# Autodesk Inventor assembly: 1.625_flex_wheel_w_versahex
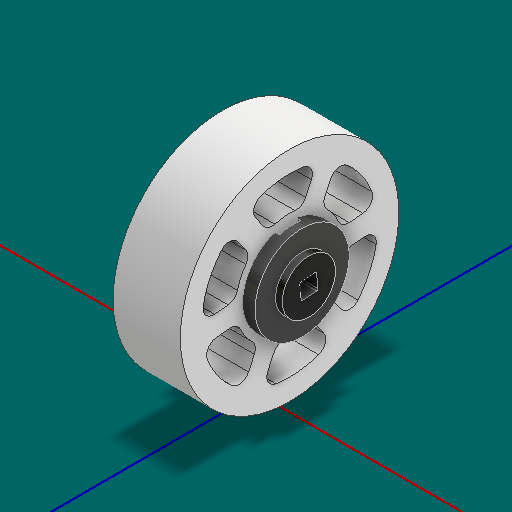
[picture p0: Inventor's stored thumbnail of the model, 512x512]
Saved by Autodesk Inventor 2025 (Build 290162000, 162)
## iProperties
Created: 2024-08-18
Part Number: 1.625_flex_wheel_w_versahex
Document SubType Name: Assembly
Designer: averey
Author: averey
## Documents named in this file (5)
- C:\Users\avere\vex_robotics_high_stakes\hardware\cad\_quick_assemblies\1.625_flex_wheel_w_versahex.iam
- C:\Users\avere\vex_robotics_high_stakes\hardware\cad\VEX-CAD-Inventor\Motion\Wheels\Flex Wheels\1.625 Flex Wheel\1.625 30A .500.ipt
- C:\Users\avere\vex_robotics_high_stakes\hardware\cad\VEX-CAD-Inventor\Motion\Wheels\Flex Wheels\1.625 Flex Wheel.ipt
- C:\Users\avere\vex_robotics_high_stakes\hardware\cad\VEX-CAD-Inventor\Motion\Wheels\Flex Wheels\VersaHex Adapters .125.ipt
- C:\Users\avere\vex_robotics_high_stakes\hardware\cad\VEX-CAD-Inventor\Motion\Insert Square.ipt
## Components (5 placed, 3 different names)
1. 1.625 30A .500:1 — Mate:1, Mate:2, Mate:3, Angle:5
2. VersaHex Adapters .125:1
3. Insert Square:1
4. VersaHex Adapters .125:2
5. Insert Square:2
## Relationships (12: Angle 5, Insert 4, Mate 3)
- [Insert]: VersaHex Adapters .125:1 ↔ Insert Square:1
- [Angle] (0 deg): VersaHex Adapters .125:1 ↔ Insert Square:1
- [Angle] (0 deg): 1.625 30A .500:1 ↔ VersaHex Adapters .125:1
- [Insert]: 1.625 30A .500:1 ↔ VersaHex Adapters .125:1
- [Insert]: VersaHex Adapters .125:2 ↔ Insert Square:2
- [Angle] (0 deg): VersaHex Adapters .125:2 ↔ Insert Square:2
- [Angle] (0 deg): 1.625 30A .500:1 ↔ VersaHex Adapters .125:2
- [Insert]: 1.625 30A .500:1 ↔ VersaHex Adapters .125:2
- Mate:1: 1.625 30A .500:1
- Mate:2 (6.35 mm): 1.625 30A .500:1
- Mate:3: 1.625 30A .500:1
- Angle:5 (0 deg): 1.625 30A .500:1
## Named parameters: d0_d5 = 0 mm, d1_d6 = 0 deg, d2_d7 = 0 deg, d9_d5 = 0 mm, d10_d6 = 0 deg
